# Autodesk Inventor assembly: Assembly6
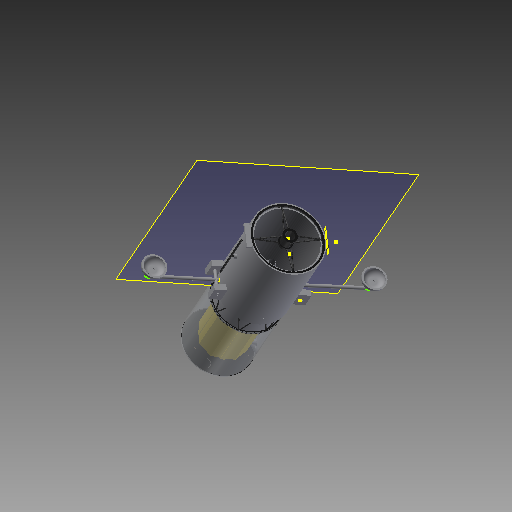
[picture p0: Inventor's stored thumbnail of the model, 512x512]
Saved by Autodesk Inventor 2018 (Build 220112000, 112)
## iProperties
Created: 2021-03-18
Part Number: Assembly6
Document SubType Name: Assembly
Designer: dell
Author: dell
## Documents named in this file (4)
- D:\Autodesk\Projects\C-C\a1\ES101 GROUP-13 PROJECT\FINAL MODEL\Resolved files\Assembly6.iam
- D:\Autodesk\Projects\C-C\a1\ES101 GROUP-13 PROJECT\FINAL MODEL\Resolved files\Assembly5.iam
- D:\Autodesk\Projects\C-C\a1\ES101 GROUP-13 PROJECT\FINAL MODEL\Resolved files\hubble.iam
- D:\Autodesk\Projects\C-C\a1\ES101 GROUP-13 PROJECT\FINAL MODEL\Resolved files\Forward Shell.iam
## Components (3 placed, 3 different names)
1. Assembly5:1 [sub-assembly] — Mate:3
2. hubble:1 [sub-assembly] — Mate:2, Mate:4
3. Forward Shell:1 [sub-assembly] — Mate:2, Mate:3, Mate:4
## Relationships (3: Mate 3)
- Mate:2: hubble:1 ↔ Forward Shell:1
- Mate:3: Assembly5:1 ↔ Forward Shell:1
- Mate:4: hubble:1 ↔ Forward Shell:1
